# Autodesk Inventor assembly: Assembly1
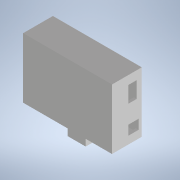
[picture p0: Inventor's stored thumbnail of the model, 180x180]
Saved by Autodesk Inventor 2021 (Build 250183000, 183)
## iProperties
Created: 2021-10-23
Part Number: Assembly1
Document SubType Name: Assembly
Designer: eddys
Author: eddys
## Documents named in this file (3)
- C:\Users\eddys\Desktop\remote switch\Assembly1.iam
- C:\Users\eddys\Desktop\remote switch\remoteswitchbox.ipt
- C:\Users\eddys\Desktop\remote switch\remoteswitchlid.ipt
## Components (2 placed, 2 different names)
1. remoteswitchbox:1 — Mate:1, Flush:1, Flush:2
2. remoteswitchlid:1 — Mate:1, Flush:1, Flush:2
## Relationships (3: Flush 2, Mate 1)
- Mate:1: remoteswitchbox:1 ↔ remoteswitchlid:1
- Flush:1: remoteswitchbox:1 ↔ remoteswitchlid:1
- Flush:2: remoteswitchbox:1 ↔ remoteswitchlid:1
